# Autodesk Inventor assembly: 2121
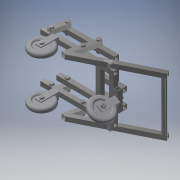
[picture p0: Inventor's stored thumbnail of the model, 180x180]
Saved by Autodesk Inventor 2019 (Build 230136000, 136)
## iProperties
Created: 2019-05-06
Part Number: 2121
Document SubType Name: Assembly
Designer: D03
Author: D03
## Documents named in this file (17)
- C:\Users\user\Desktop\2121.iam
- C:\Users\user\Desktop\新增資料夾\1.ipt
- C:\Users\user\Desktop\新增資料夾\7.ipt
- C:\Users\user\Desktop\新增資料夾\6.ipt
- C:\Users\user\Desktop\新增資料夾\4.ipt
- C:\Users\user\Desktop\新增資料夾\3.ipt
- C:\Users\user\Desktop\新增資料夾\9.ipt
- C:\Users\user\Desktop\新增資料夾\CNS 150 - A - 2.2.ipt
- C:\Users\user\Desktop\新增資料夾\CNS 3128 - M 2 x 0.4.ipt
- C:\Users\user\Desktop\新增資料夾\輪子架.ipt
- C:\Users\user\Desktop\新增資料夾\輪子.ipt
- C:\Users\user\Desktop\新增資料夾\CNS 3121 - M2 x 12.ipt
- C:\Users\user\Desktop\新增資料夾\CNS 3121 - M2 x 12-2.ipt
- C:\Users\user\Desktop\新增資料夾\後輪架.ipt
- C:\Users\user\Desktop\新增資料夾\鉚釘.ipt
- C:\Users\user\Desktop\新增資料夾\支架.ipt
- C:\Users\user\Desktop\新增資料夾\2-1.ipt
## Components (70 placed, 16 different names)
1. 1:1 — 插入:2, 插入:9, 插入:21, 插入:22, 齊平:4, 貼合:25, 齊平:5, 貼合:45, 齊平:13, 齊平:17, 齊平:18, 貼合:53, 齊平:21
2. 1:2 — 插入:4, 插入:11, 插入:14, 插入:25, 貼合:27, 齊平:8, 齊平:14, 貼合:46, 貼合:49
3. 3:1 — 插入:6, 插入:10, 插入:13, 插入:24, 貼合:47, 對稱:1, 齊平:22, 齊平:23
4. 3:2 — 插入:7, 插入:8, 插入:20, 插入:23, 貼合:48, 齊平:15, 齊平:16, 對稱:1
5. 4:1 — 插入:2, 插入:7, 插入:18, 插入:19
6. 4:2 — 插入:4, 插入:6, 插入:12, 插入:15
7. 6:1 — 貼合:17, 貼合:18, 貼合:19, 齊平:2, 貼合:22, 齊平:3, 齊平:24
8. 6:2 — 貼合:14, 貼合:15, 貼合:16, 貼合:21, 齊平:24
9. 7:1 — 貼合:20, 貼合:21, 貼合:22, 貼合:23
10. 9:1 — 貼合:14, 貼合:15, 貼合:16, 插入:8, 插入:9, 插入:16, 插入:17
11. 9:2 — 貼合:17, 貼合:18, 貼合:19, 插入:10, 插入:11, 插入:26, 插入:27
12. CNS 150 - A - 2.2:1 — 插入:15, 插入:50
13. CNS 150 - A - 2.2:2 — 插入:12, 插入:51
14. CNS 150 - A - 2.2:3 — 插入:24, 插入:36
15. CNS 150 - A - 2.2:4 — 插入:25, 插入:38
16. CNS 150 - A - 2.2:5 — 插入:20, 插入:40
17. CNS 150 - A - 2.2:6 — 插入:21, 插入:41
18. CNS 150 - A - 2.2:7 — 插入:19, 插入:52
19. CNS 150 - A - 2.2:8 — 插入:18, 插入:53
20. CNS 150 - A - 2.2:9 — 插入:26, 插入:48
21. CNS 150 - A - 2.2:10 — 插入:14, 插入:39
22. CNS 150 - A - 2.2:11 — 插入:27, 插入:49
23. CNS 150 - A - 2.2:12 — 插入:13, 插入:37
24. CNS 150 - A - 2.2:13 — 插入:23, 插入:43
25. CNS 150 - A - 2.2:14 — 插入:22, 插入:42
26. CNS 150 - A - 2.2:15 — 插入:17, 插入:54
27. CNS 150 - A - 2.2:16 — 插入:16, 插入:55
28. CNS 3128 - M 2 x 0.4:2 — 插入:39
29. CNS 3128 - M 2 x 0.4:3 — 插入:38
30. CNS 3128 - M 2 x 0.4:4 — 插入:37
31. CNS 3128 - M 2 x 0.4:5 — 插入:36
32. CNS 3128 - M 2 x 0.4:6 — 插入:42
33. CNS 3128 - M 2 x 0.4:7 — 插入:41
34. CNS 3128 - M 2 x 0.4:8 — 插入:43
35. CNS 3128 - M 2 x 0.4:9 — 插入:40
36. 輪子架:1 — 貼合:25, 貼合:26, 齊平:6, 貼合:29, 貼合:35, 插入:44, 插入:45
37. 輪子架:2 — 齊平:7, 貼合:27, 齊平:9, 貼合:31, 貼合:36, 插入:46, 插入:47
38. 輪子:1 — 貼合:28, 貼合:35
39. 輪子:2 — 貼合:30, 貼合:36
40. CNS 150 - A - 2.2:17 — 插入:44, 插入:59
41. CNS 150 - A - 2.2:19 — 插入:47, 插入:58
42. CNS 150 - A - 2.2:20 — 插入:46, 插入:56
43. CNS 150 - A - 2.2:21 — 插入:45, 插入:57
44. CNS 3121 - M2 x 12:1 — 插入:55
45. CNS 3121 - M2 x 12:2 — 插入:54
46. CNS 3121 - M2 x 12:3 — 插入:53
47. CNS 3121 - M2 x 12:4 — 插入:52
48. CNS 3121 - M2 x 12:5 — 插入:50
49. CNS 3121 - M2 x 12:6 — 插入:51
50. CNS 3121 - M2 x 12:7 — 插入:49
51. CNS 3121 - M2 x 12:8 — 插入:48
52. CNS 3128 - M 2 x 0.4:11 — 插入:58
53. CNS 3128 - M 2 x 0.4:12 — 插入:59
54. CNS 3121 - M2 x 12-2:1 — 插入:57
55. CNS 3121 - M2 x 12-2:2 — 插入:56
56. 後輪架:1 — 插入:60, 插入:66, 齊平:10, 貼合:50, 貼合:51, 齊平:19, 齊平:20
57. 輪子架:3 — 插入:60, 貼合:41, 貼合:43, 插入:61, 插入:62, 貼合:44, 插入:65
58. 輪子:3 — 貼合:40, 貼合:43
59. CNS 3128 - M 2 x 0.4:13 — 插入:64
60. CNS 3121 - M2 x 12-2:3 — 插入:63
61. CNS 150 - A - 2.2:22 — 插入:61, 插入:63
62. CNS 150 - A - 2.2:23 — 插入:62, 插入:64
63. 鉚釘:1 — 貼合:44, 插入:65
64. CNS 150 - A - 2.2:24 — 插入:66, 插入:67
65. CNS 3128 - M 2 x 0.4:14 — 插入:67
66. 支架:1 — 齊平:12, 齊平:14, 貼合:46
67. 支架:2 — 齊平:11, 貼合:45, 齊平:13
68. 2-1:2 — 貼合:47, 貼合:48, 齊平:15, 齊平:16, 齊平:22, 齊平:23, 齊平:26
69. 2-1:3 — 齊平:17, 齊平:18, 貼合:49, 貼合:50, 貼合:51
70. 2-1:4 — 貼合:53, 齊平:20, 齊平:21
## Relationships (119: Insert 56, Mate 38, Flush 24, Symmetry 1)
- 插入:2 [Insert]: 1:1 ↔ 4:1
- 插入:4 [Insert]: 1:2 ↔ 4:2
- 插入:6 [Insert]: 3:1 ↔ 4:2
- 插入:7 [Insert]: 3:2 ↔ 4:1
- 貼合:14 [Mate]: 6:2 ↔ 9:1
- 貼合:15 [Mate]: 6:2 ↔ 9:1
- 貼合:16 [Mate]: 6:2 ↔ 9:1
- 貼合:17 [Mate]: 6:1 ↔ 9:2
- 貼合:18 [Mate]: 6:1 ↔ 9:2
- 貼合:19 [Mate]: 6:1 ↔ 9:2
- 齊平:2 [Flush] (-3 mm): 6:1
- 貼合:20 [Mate]: 7:1
- 貼合:21 [Mate]: 6:2 ↔ 7:1
- 貼合:22 [Mate]: 6:1 ↔ 7:1
- 齊平:3 [Flush] (-2.5 mm): 6:1
- 貼合:23 [Mate]: 7:1
- 貼合:24 [Mate]
- 插入:8 [Insert]: 3:2 ↔ 9:1
- 插入:9 [Insert]: 1:1 ↔ 9:1
- 插入:10 [Insert]: 3:1 ↔ 9:2
- 插入:11 [Insert]: 1:2 ↔ 9:2
- 插入:12 [Insert]: 4:2 ↔ CNS 150 - A - 2.2:2
- 插入:13 [Insert]: 3:1 ↔ CNS 150 - A - 2.2:12
- 插入:14 [Insert]: 1:2 ↔ CNS 150 - A - 2.2:10
- 插入:15 [Insert]: 4:2 ↔ CNS 150 - A - 2.2:1
- 插入:16 [Insert]: 9:1 ↔ CNS 150 - A - 2.2:16
- 插入:17 [Insert]: 9:1 ↔ CNS 150 - A - 2.2:15
- 插入:18 [Insert]: 4:1 ↔ CNS 150 - A - 2.2:8
- 插入:19 [Insert]: 4:1 ↔ CNS 150 - A - 2.2:7
- 插入:20 [Insert]: 3:2 ↔ CNS 150 - A - 2.2:5
- 插入:21 [Insert]: 1:1 ↔ CNS 150 - A - 2.2:6
- 插入:22 [Insert]: 1:1 ↔ CNS 150 - A - 2.2:14
- 插入:23 [Insert]: 3:2 ↔ CNS 150 - A - 2.2:13
- 插入:24 [Insert]: 3:1 ↔ CNS 150 - A - 2.2:3
- 插入:25 [Insert]: 1:2 ↔ CNS 150 - A - 2.2:4
- 插入:26 [Insert]: 9:2 ↔ CNS 150 - A - 2.2:9
- 插入:27 [Insert]: 9:2 ↔ CNS 150 - A - 2.2:11
- 插入:36 [Insert]: CNS 150 - A - 2.2:3 ↔ CNS 3128 - M 2 x 0.4:5
- 插入:37 [Insert]: CNS 150 - A - 2.2:12 ↔ CNS 3128 - M 2 x 0.4:4
- 插入:38 [Insert]: CNS 150 - A - 2.2:4 ↔ CNS 3128 - M 2 x 0.4:3
- 插入:39 [Insert]: CNS 150 - A - 2.2:10 ↔ CNS 3128 - M 2 x 0.4:2
- 插入:40 [Insert]: CNS 150 - A - 2.2:5 ↔ CNS 3128 - M 2 x 0.4:9
- 插入:41 [Insert]: CNS 150 - A - 2.2:6 ↔ CNS 3128 - M 2 x 0.4:7
- 插入:42 [Insert]: CNS 150 - A - 2.2:14 ↔ CNS 3128 - M 2 x 0.4:6
- 插入:43 [Insert]: CNS 150 - A - 2.2:13 ↔ CNS 3128 - M 2 x 0.4:8
- 齊平:4 [Flush] (-1 mm): 1:1
- 貼合:25 [Mate]: 1:1 ↔ 輪子架:1
- 貼合:26 [Mate]: 輪子架:1
- 齊平:5 [Flush] (-14 mm): 1:1
- 齊平:6 [Flush]: 輪子架:1
- 齊平:7 [Flush]: 輪子架:2
- 貼合:27 [Mate]: 1:2 ↔ 輪子架:2
- 齊平:8 [Flush] (-4 mm): 1:2
- 齊平:9 [Flush]: 輪子架:2
- 貼合:28 [Mate]: 輪子:1
- 貼合:29 [Mate]: 輪子架:1
- 貼合:30 [Mate]: 輪子:2
- 貼合:31 [Mate]: 輪子架:2
- 貼合:32 [Mate]
- 貼合:33 [Mate]
- 貼合:34 [Mate]
- 貼合:35 [Mate]: 輪子架:1 ↔ 輪子:1
- 貼合:36 [Mate]: 輪子架:2 ↔ 輪子:2
- 插入:44 [Insert]: 輪子架:1 ↔ CNS 150 - A - 2.2:17
- 插入:45 [Insert]: 輪子架:1 ↔ CNS 150 - A - 2.2:21
- 插入:46 [Insert]: 輪子架:2 ↔ CNS 150 - A - 2.2:20
- 插入:47 [Insert]: 輪子架:2 ↔ CNS 150 - A - 2.2:19
- 插入:48 [Insert]: CNS 150 - A - 2.2:9 ↔ CNS 3121 - M2 x 12:8
- 插入:49 [Insert]: CNS 150 - A - 2.2:11 ↔ CNS 3121 - M2 x 12:7
- 插入:50 [Insert]: CNS 150 - A - 2.2:1 ↔ CNS 3121 - M2 x 12:5
- 插入:51 [Insert]: CNS 150 - A - 2.2:2 ↔ CNS 3121 - M2 x 12:6
- 插入:52 [Insert]: CNS 150 - A - 2.2:7 ↔ CNS 3121 - M2 x 12:4
- 插入:53 [Insert]: CNS 150 - A - 2.2:8 ↔ CNS 3121 - M2 x 12:3
- 插入:54 [Insert]: CNS 150 - A - 2.2:15 ↔ CNS 3121 - M2 x 12:2
- 插入:55 [Insert]: CNS 150 - A - 2.2:16 ↔ CNS 3121 - M2 x 12:1
- 插入:56 [Insert]: CNS 150 - A - 2.2:20 ↔ CNS 3121 - M2 x 12-2:2
- 插入:57 [Insert]: CNS 150 - A - 2.2:21 ↔ CNS 3121 - M2 x 12-2:1
- 插入:58 [Insert]: CNS 150 - A - 2.2:19 ↔ CNS 3128 - M 2 x 0.4:11
- 插入:59 [Insert]: CNS 150 - A - 2.2:17 ↔ CNS 3128 - M 2 x 0.4:12
- 插入:60 [Insert]: 後輪架:1 ↔ 輪子架:3
- 貼合:40 [Mate]: 輪子:3
- 貼合:41 [Mate]: 輪子架:3
- 貼合:42 [Mate]
- 貼合:43 [Mate]: 輪子架:3 ↔ 輪子:3
- 插入:61 [Insert]: 輪子架:3 ↔ CNS 150 - A - 2.2:22
- 插入:62 [Insert]: 輪子架:3 ↔ CNS 150 - A - 2.2:23
- 插入:63 [Insert]: CNS 3121 - M2 x 12-2:3 ↔ CNS 150 - A - 2.2:22
- 插入:64 [Insert]: CNS 3128 - M 2 x 0.4:13 ↔ CNS 150 - A - 2.2:23
- 貼合:44 [Mate]: 輪子架:3 ↔ 鉚釘:1
- 插入:65 [Insert]: 輪子架:3 ↔ 鉚釘:1
- 插入:66 [Insert]: 後輪架:1 ↔ CNS 150 - A - 2.2:24
- 插入:67 [Insert]: CNS 150 - A - 2.2:24 ↔ CNS 3128 - M 2 x 0.4:14
- 齊平:10 [Flush] (-8.5 mm): 後輪架:1
- 齊平:11 [Flush]: 支架:2
- 齊平:12 [Flush]: 支架:1
- 貼合:45 [Mate]: 1:1 ↔ 支架:2
- 齊平:13 [Flush]: 1:1 ↔ 支架:2
- 齊平:14 [Flush]: 1:2 ↔ 支架:1
- 貼合:46 [Mate]: 1:2 ↔ 支架:1
- 貼合:47 [Mate]: 3:1 ↔ 2-1:2
- 貼合:48 [Mate]: 3:2 ↔ 2-1:2
- 齊平:15 [Flush]: 3:2 ↔ 2-1:2
- 齊平:16 [Flush]: 3:2 ↔ 2-1:2
- 齊平:17 [Flush]: 1:1 ↔ 2-1:3
- 齊平:18 [Flush]: 1:1 ↔ 2-1:3
- 貼合:49 [Mate]: 1:2 ↔ 2-1:3
- 貼合:50 [Mate]: 後輪架:1 ↔ 2-1:3
- 貼合:51 [Mate]: 後輪架:1 ↔ 2-1:3
- 對稱:1 [Symmetry]: 3:1 ↔ 3:2
- 齊平:19 [Flush] (-11 mm): 後輪架:1
- 貼合:52 [Mate]
- 貼合:53 [Mate]: 1:1 ↔ 2-1:4
- 齊平:20 [Flush]: 後輪架:1 ↔ 2-1:4
- 齊平:21 [Flush]: 1:1 ↔ 2-1:4
- 齊平:22 [Flush]: 3:1 ↔ 2-1:2
- 齊平:23 [Flush]: 3:1 ↔ 2-1:2
- 齊平:24 [Flush]: 6:1 ↔ 6:2
- 貼合:55 [Mate]
- 齊平:26 [Flush] (-2.5 mm): 2-1:2
## Named parameters: sa_0 = 3186.56, sa_1 = -19744.5, sa_2 = -3.8e-11
note: some values were not read from the file. Shown as the stored number, unit unknown: "sa_0", "sa_1", "sa_2".
